# Autodesk Inventor assembly: 2-4
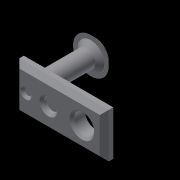
[picture p0: Inventor's stored thumbnail of the model, 180x180]
Saved by Autodesk Inventor 2017 (Build 210142000, 142)
## iProperties
Part Number: 2-4
Material: 一般
Document SubType Name: Assembly
Designer: r0909
Author: r0909
## Documents named in this file (4)
- C:\Users\r0909\Desktop\2-4.iam
- C:\Users\r0909\Desktop\2-1.ipt
- C:\Users\r0909\Desktop\2-2.ipt
- C:\Users\r0909\Desktop\2-3.ipt
## Components (3 placed, 3 different names)
1. 2-1:1 — 齊平:1, 貼合:1, 貼合:2, 貼合:3, 貼合:4, 貼合:5
2. 2-2:1 — 貼合:2, 貼合:3
3. 2-3:1 — 貼合:4, 貼合:5
## Relationships (6: Mate 5, Flush 1)
- 齊平:1 [Flush]: 2-1:1
- 貼合:1 [Mate]: 2-1:1
- 貼合:2 [Mate]: 2-1:1 ↔ 2-2:1
- 貼合:3 [Mate]: 2-1:1 ↔ 2-2:1
- 貼合:4 [Mate]: 2-1:1 ↔ 2-3:1
- 貼合:5 [Mate]: 2-1:1 ↔ 2-3:1
